# Autodesk Inventor assembly: MK4i Master Structure
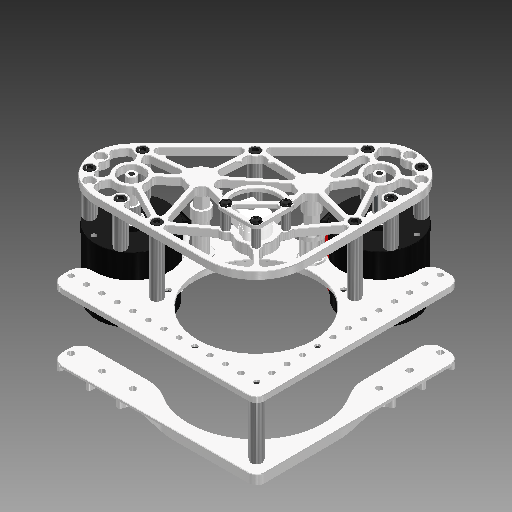
[picture p0: Inventor's stored thumbnail of the model, 512x512]
Saved by Autodesk Inventor 2025 (Build 290162010, 162A)
## iProperties
Created: 2024-07-14
Part Number: MK4i Master Structure
Document SubType Name: Assembly
Designer: rohan
Author: rohan
## Documents named in this file (24)
- D:\ultimate-hecker\Computer-Aided-Design\FRC-Offseason-Design-Training\Parts Library\Drivetrains\Swerve Modules\MK4i\MK4i Master Structure.iam
- D:\ultimate-hecker\Computer-Aided-Design\FRC-Offseason-Design-Training\Parts Library\Drivetrains\Swerve Modules\MK4i\MK4i Wheel Guard.ipt
- D:\ultimate-hecker\Computer-Aided-Design\FRC-Offseason-Design-Training\Parts Library\Drivetrains\Swerve Modules\MK4i\MK4i Motor Mount.ipt
- D:\ultimate-hecker\Computer-Aided-Design\FRC-Offseason-Design-Training\Parts Library\Drivetrains\Swerve Modules\MK4i\MK4i Midsection.ipt
- D:\ultimate-hecker\Computer-Aided-Design\FRC-Offseason-Design-Training\Parts Library\Hardware\Spacers\Spacers & Standoffs\Aluminum Unthreaded Spacer (No. 10 x 1.875Lg x 0.375OD).ipt
- D:\ultimate-hecker\Computer-Aided-Design\FRC-Offseason-Design-Training\Parts Library\Hardware\Spacers\Spacers & Standoffs.ipt
- D:\ultimate-hecker\Computer-Aided-Design\FRC-Offseason-Design-Training\Parts Library\Hardware\Spacers\Spacers & Standoffs\Aluminum Unthreaded Spacer (No. 10 x 1.125Lg x 0.375OD).ipt
- D:\ultimate-hecker\Computer-Aided-Design\FRC-Offseason-Design-Training\Parts Library\Motors\FRC\NEO.ipt
- D:\ultimate-hecker\Computer-Aided-Design\FRC-Offseason-Design-Training\Parts Library\Hardware\Fasteners\Machine Screws\10-32 UNFx1.5 Socket Head Cap Screw.ipt
- D:\ultimate-hecker\Computer-Aided-Design\FRC-Offseason-Design-Training\Parts Library\Hardware\Fasteners\Machine Screws.ipt
- D:\ultimate-hecker\Computer-Aided-Design\FRC-Offseason-Design-Training\Parts Library\Hardware\Fasteners\Machine Screws\10-32 UNFx2.25 Socket Head Cap Screw.ipt
- D:\ultimate-hecker\Computer-Aided-Design\FRC-Offseason-Design-Training\Parts Library\Hardware\Spacers\Spacers & Standoffs\Aluminum Threaded Standoff (8x32 x 0.563Lg x 0.25OD).ipt
- D:\ultimate-hecker\Computer-Aided-Design\FRC-Offseason-Design-Training\Parts Library\Drivetrains\Swerve Modules\MK4i\MK4i Encoder Cover.ipt
- D:\ultimate-hecker\Computer-Aided-Design\FRC-Offseason-Design-Training\Parts Library\Hardware\Spacers\Spacers & Standoffs\SDS Neo Shaft Spacer 0.437.ipt
- D:\ultimate-hecker\Computer-Aided-Design\FRC-Offseason-Design-Training\Parts Library\Hardware\Spacers\Spacers & Standoffs\SDS Neo Shaft Spacer 1mm.ipt
- D:\ultimate-hecker\Computer-Aided-Design\FRC-Offseason-Design-Training\Parts Library\Electronics\FRC\Sensors\CTRE Mag Encoder.ipt
- D:\ultimate-hecker\Computer-Aided-Design\FRC-Offseason-Design-Training\Parts Library\Hardware\Fasteners\Machine Screws\8-32 UNCx0.875 Button Head Cap Screw.ipt
- D:\ultimate-hecker\Computer-Aided-Design\FRC-Offseason-Design-Training\Parts Library\Power Transfer\Bearings and Bushings\Bearings\688 Bearing.ipt
- D:\ultimate-hecker\Computer-Aided-Design\FRC-Offseason-Design-Training\Parts Library\Power Transfer\Bearings and Bushings\Bearings\R188ZZ Bearing.ipt
- D:\ultimate-hecker\Computer-Aided-Design\FRC-Offseason-Design-Training\Parts Library\Drivetrains\Swerve Modules\MK4i\MK4i Drive Shaft Idler.ipt
- D:\ultimate-hecker\Computer-Aided-Design\FRC-Offseason-Design-Training\Parts Library\Drivetrains\Swerve Modules\MK4i\MK4i Steering Shaft.ipt
- D:\ultimate-hecker\Computer-Aided-Design\FRC-Offseason-Design-Training\Parts Library\Hardware\Fasteners\Machine Screws\10-32 UNFx0.25 Button Head Cap Screw.ipt
- D:\ultimate-hecker\Computer-Aided-Design\FRC-Offseason-Design-Training\Parts Library\Drivetrains\Swerve Modules\MK4i\MK4i Steering Shaft Spacer.ipt
- D:\ultimate-hecker\Computer-Aided-Design\FRC-Offseason-Design-Training\Parts Library\Hardware\Fasteners\Machine Key, 2 X 2 X 12mm.ipt
## Components (49 placed, 21 different names)
1. MK4i Wheel Guard:1 — Insert:1, Insert:25, Flush:1
2. MK4i Motor Mount:1 — Insert:5, Insert:6, Insert:7, Insert:8, Insert:9, Insert:10, Insert:11, Insert:12, Insert:17, Insert:18, Insert:19, Insert:20, Insert:21, Insert:22, Insert:23, Insert:24, Insert:26, Insert:27, Insert:28, Insert:33, Insert:34, Insert:41, Insert:42, Insert:45
3. MK4i Midsection:1 — Insert:2, Insert:3, Insert:4, Insert:38, Insert:39, Insert:44, Insert:46, Insert:47, Insert:48, Insert:49, Insert:50, Flush:1
4. Aluminum Unthreaded Spacer (No. 10 x 1.875Lg x 0.375OD):1 — Insert:1, Insert:2
5. Aluminum Unthreaded Spacer (No. 10 x 1.875Lg x 0.375OD):2 — Insert:3, Insert:5
6. Aluminum Unthreaded Spacer (No. 10 x 1.875Lg x 0.375OD):3 — Insert:4, Insert:6
7. Aluminum Unthreaded Spacer (No. 10 x 1.125Lg x 0.375OD):4 — Insert:11, Insert:14
8. Aluminum Unthreaded Spacer (No. 10 x 1.125Lg x 0.375OD):5 — Insert:7, Insert:16
9. Aluminum Unthreaded Spacer (No. 10 x 1.125Lg x 0.375OD):6 — Insert:8
10. Aluminum Unthreaded Spacer (No. 10 x 1.125Lg x 0.375OD):7 — Insert:9, Insert:15
11. Aluminum Unthreaded Spacer (No. 10 x 1.125Lg x 0.375OD):8 — Insert:10
12. Aluminum Unthreaded Spacer (No. 10 x 1.125Lg x 0.375OD):9 — Insert:12, Insert:13
13. NEO:1 — Insert:15, Insert:16, Insert:31, Mate:4, Mate:5
14. NEO:2 — Insert:13, Insert:14, Insert:32, Mate:1, Mate:2, Mate:3
15. 10-32 UNFx1.5 Socket Head Cap Screw:1 — Insert:20
16. 10-32 UNFx1.5 Socket Head Cap Screw:2 — Insert:18
17. 10-32 UNFx1.5 Socket Head Cap Screw:3 — Insert:17
18. 10-32 UNFx1.5 Socket Head Cap Screw:4 — Insert:22
19. 10-32 UNFx1.5 Socket Head Cap Screw:5 — Insert:21
20. 10-32 UNFx1.5 Socket Head Cap Screw:6 — Insert:19
21. 10-32 UNFx2.25 Socket Head Cap Screw:7 — Insert:25
22. 10-32 UNFx2.25 Socket Head Cap Screw:8 — Insert:24
23. 10-32 UNFx2.25 Socket Head Cap Screw:9 — Insert:23
24. Aluminum Threaded Standoff (8x32 x 0.563Lg x 0.25OD):12 — Insert:26, Insert:29
25. Aluminum Threaded Standoff (8x32 x 0.563Lg x 0.25OD):13 — Insert:28
26. Aluminum Threaded Standoff (8x32 x 0.563Lg x 0.25OD):14 — Insert:27, Insert:30
27. MK4i Encoder Cover:1 — Insert:29, Insert:30, Insert:35, Insert:36, Insert:37
28. SDS Neo Shaft Spacer 0.437:15 — Insert:31, Tangent:1
29. SDS Neo Shaft Spacer 1mm:16 — Insert:32
30. CTRE Mag Encoder:1 — Insert:33, Insert:34
31. 8-32 UNCx0.875 Button Head Cap Screw:10 — Insert:37
32. 8-32 UNCx0.875 Button Head Cap Screw:11 — Insert:36
33. 8-32 UNCx0.875 Button Head Cap Screw:12 — Insert:35
34. 688 Bearing:1 — Insert:38, Insert:40
35. R188ZZ Bearing:1 — Insert:39, Insert:43
36. MK4i Drive Shaft Idler:1 — Insert:40
37. 688 Bearing:2 — Insert:41, Insert:51
38. 688 Bearing:3 — Insert:42
39. MK4i Steering Shaft:1 — Insert:43
40. Aluminum Unthreaded Spacer (No. 10 x 1.875Lg x 0.375OD):17 — Insert:44
41. 10-32 UNFx2.25 Socket Head Cap Screw:13 — Insert:45
42. 10-32 UNFx0.25 Button Head Cap Screw:14 — Insert:46
43. 10-32 UNFx0.25 Button Head Cap Screw:15 — Insert:47
44. 10-32 UNFx0.25 Button Head Cap Screw:16 — Insert:50
45. 10-32 UNFx0.25 Button Head Cap Screw:17 — Insert:49
46. 10-32 UNFx0.25 Button Head Cap Screw:18 — Insert:48
47. MK4i Steering Shaft Spacer:1 — Insert:51
48. Machine Key, 2 X 2 X 12mm:1 — Mate:1, Mate:2, Mate:3
49. Machine Key, 2 X 2 X 12mm:2 — Mate:4, Mate:5, Tangent:1
## Relationships (58: Insert 51, Mate 5, Tangent 1, Flush 1)
- Insert:1: MK4i Wheel Guard:1 ↔ Aluminum Unthreaded Spacer (No. 10 x 1.875Lg x 0.375OD):1
- Insert:2: MK4i Midsection:1 ↔ Aluminum Unthreaded Spacer (No. 10 x 1.875Lg x 0.375OD):1
- Insert:3: MK4i Midsection:1 ↔ Aluminum Unthreaded Spacer (No. 10 x 1.875Lg x 0.375OD):2
- Insert:4: MK4i Midsection:1 ↔ Aluminum Unthreaded Spacer (No. 10 x 1.875Lg x 0.375OD):3
- Insert:5: MK4i Motor Mount:1 ↔ Aluminum Unthreaded Spacer (No. 10 x 1.875Lg x 0.375OD):2
- Insert:6: MK4i Motor Mount:1 ↔ Aluminum Unthreaded Spacer (No. 10 x 1.875Lg x 0.375OD):3
- Insert:7: MK4i Motor Mount:1 ↔ Aluminum Unthreaded Spacer (No. 10 x 1.125Lg x 0.375OD):5
- Insert:8: MK4i Motor Mount:1 ↔ Aluminum Unthreaded Spacer (No. 10 x 1.125Lg x 0.375OD):6
- Insert:9: MK4i Motor Mount:1 ↔ Aluminum Unthreaded Spacer (No. 10 x 1.125Lg x 0.375OD):7
- Insert:10: MK4i Motor Mount:1 ↔ Aluminum Unthreaded Spacer (No. 10 x 1.125Lg x 0.375OD):8
- Insert:11: MK4i Motor Mount:1 ↔ Aluminum Unthreaded Spacer (No. 10 x 1.125Lg x 0.375OD):4
- Insert:12: MK4i Motor Mount:1 ↔ Aluminum Unthreaded Spacer (No. 10 x 1.125Lg x 0.375OD):9
- Insert:13: Aluminum Unthreaded Spacer (No. 10 x 1.125Lg x 0.375OD):9 ↔ NEO:2
- Insert:14: Aluminum Unthreaded Spacer (No. 10 x 1.125Lg x 0.375OD):4 ↔ NEO:2
- Insert:15: Aluminum Unthreaded Spacer (No. 10 x 1.125Lg x 0.375OD):7 ↔ NEO:1
- Insert:16: Aluminum Unthreaded Spacer (No. 10 x 1.125Lg x 0.375OD):5 ↔ NEO:1
- Insert:17: MK4i Motor Mount:1 ↔ 10-32 UNFx1.5 Socket Head Cap Screw:3
- Insert:18: MK4i Motor Mount:1 ↔ 10-32 UNFx1.5 Socket Head Cap Screw:2
- Insert:19: MK4i Motor Mount:1 ↔ 10-32 UNFx1.5 Socket Head Cap Screw:6
- Insert:20: MK4i Motor Mount:1 ↔ 10-32 UNFx1.5 Socket Head Cap Screw:1
- Insert:21: MK4i Motor Mount:1 ↔ 10-32 UNFx1.5 Socket Head Cap Screw:5
- Insert:22: MK4i Motor Mount:1 ↔ 10-32 UNFx1.5 Socket Head Cap Screw:4
- Insert:23: MK4i Motor Mount:1 ↔ 10-32 UNFx2.25 Socket Head Cap Screw:9
- Insert:24: MK4i Motor Mount:1 ↔ 10-32 UNFx2.25 Socket Head Cap Screw:8
- Insert:25: MK4i Wheel Guard:1 ↔ 10-32 UNFx2.25 Socket Head Cap Screw:7
- Insert:26: MK4i Motor Mount:1 ↔ Aluminum Threaded Standoff (8x32 x 0.563Lg x 0.25OD):12
- Insert:27: MK4i Motor Mount:1 ↔ Aluminum Threaded Standoff (8x32 x 0.563Lg x 0.25OD):14
- Insert:28: MK4i Motor Mount:1 ↔ Aluminum Threaded Standoff (8x32 x 0.563Lg x 0.25OD):13
- Insert:29: Aluminum Threaded Standoff (8x32 x 0.563Lg x 0.25OD):12 ↔ MK4i Encoder Cover:1
- Insert:30: Aluminum Threaded Standoff (8x32 x 0.563Lg x 0.25OD):14 ↔ MK4i Encoder Cover:1
- Insert:31: NEO:1 ↔ SDS Neo Shaft Spacer 0.437:15
- Insert:32: NEO:2 ↔ SDS Neo Shaft Spacer 1mm:16
- Insert:33: MK4i Motor Mount:1 ↔ CTRE Mag Encoder:1
- Insert:34: MK4i Motor Mount:1 ↔ CTRE Mag Encoder:1
- Insert:35: MK4i Encoder Cover:1 ↔ 8-32 UNCx0.875 Button Head Cap Screw:12
- Insert:36: MK4i Encoder Cover:1 ↔ 8-32 UNCx0.875 Button Head Cap Screw:11
- Insert:37: MK4i Encoder Cover:1 ↔ 8-32 UNCx0.875 Button Head Cap Screw:10
- Insert:38: MK4i Midsection:1 ↔ 688 Bearing:1
- Insert:39: MK4i Midsection:1 ↔ R188ZZ Bearing:1
- Insert:40: 688 Bearing:1 ↔ MK4i Drive Shaft Idler:1
- Insert:41: MK4i Motor Mount:1 ↔ 688 Bearing:2
- Insert:42: MK4i Motor Mount:1 ↔ 688 Bearing:3
- Insert:43: R188ZZ Bearing:1 ↔ MK4i Steering Shaft:1
- Insert:44: MK4i Midsection:1 ↔ Aluminum Unthreaded Spacer (No. 10 x 1.875Lg x 0.375OD):17
- Insert:45: MK4i Motor Mount:1 ↔ 10-32 UNFx2.25 Socket Head Cap Screw:13
- Insert:46: MK4i Midsection:1 ↔ 10-32 UNFx0.25 Button Head Cap Screw:14
- Insert:47: MK4i Midsection:1 ↔ 10-32 UNFx0.25 Button Head Cap Screw:15
- Insert:48: MK4i Midsection:1 ↔ 10-32 UNFx0.25 Button Head Cap Screw:18
- Insert:49: MK4i Midsection:1 ↔ 10-32 UNFx0.25 Button Head Cap Screw:17
- Insert:50: MK4i Midsection:1 ↔ 10-32 UNFx0.25 Button Head Cap Screw:16
- Insert:51: 688 Bearing:2 ↔ MK4i Steering Shaft Spacer:1
- Mate:1: NEO:2 ↔ Machine Key, 2 X 2 X 12mm:1
- Mate:2: NEO:2 ↔ Machine Key, 2 X 2 X 12mm:1
- Mate:3: NEO:2 ↔ Machine Key, 2 X 2 X 12mm:1
- Mate:4: NEO:1 ↔ Machine Key, 2 X 2 X 12mm:2
- Mate:5: NEO:1 ↔ Machine Key, 2 X 2 X 12mm:2
- Tangent:1: SDS Neo Shaft Spacer 0.437:15 ↔ Machine Key, 2 X 2 X 12mm:2
- Flush:1: MK4i Wheel Guard:1 ↔ MK4i Midsection:1
